# Autodesk Inventor assembly: FE-100 Main Section
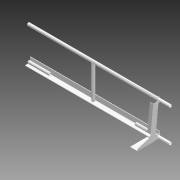
[picture p0: Inventor's stored thumbnail of the model, 180x180]
Saved by Autodesk Inventor 2021 (Build 250183000, 183)
## iProperties
Created: 2021-01-11
Part Number: FE-100 Main Section
Document SubType Name: Assembly
## Documents named in this file (7)
- D:\FIRST\Design\FRC Fields\Generic Field Base\FE-100 Side Wall\FE-110 Main Section\FE-100 Main Section.iam
- D:\FIRST\Design\FRC Fields\Generic Field Base\FE-100 Side Wall\FE-110 Main Section\FE-110-001 Floor L Section.ipt
- D:\FIRST\Design\FRC Fields\Generic Field Base\FE-100 Side Wall\FE-110 Main Section\FE-110-002 Upright Middle Section.ipt
- D:\FIRST\Design\FRC Fields\Generic Field Base\FE-100 Side Wall\FE-110 Main Section\FE-110-003 Top Bar.ipt
- D:\FIRST\Design\FRC Fields\Generic Field Base\FE-100 Side Wall\FE-110 Main Section\FE-110-004 Bottom Side Bar.ipt
- D:\FIRST\Design\FRC Fields\Generic Field Base\FE-100 Side Wall\FE-110 Main Section\FE-110-005 Inside Connector Bar.ipt
- D:\FIRST\Design\FRC Fields\Generic Field Base\FE-100 Side Wall\FE-110 Main Section\FE-110-006 Side Holder.ipt
## Components (8 placed, 6 different names)
1. FE-110-001 Floor L Section:1 — Tangent:1, Mate:2, Flush:1, Angle:1, Tangent:2, Flush:2, Tangent:3, Flush:4
2. FE-110-002 Upright Middle Section:1 — Mate:1, Tangent:1, Mate:2, Mate:3
3. FE-110-003 Top Bar:1 — Mate:3, Flush:1, Angle:1, Mate:4, Flush:3, Mate:5, Mate:6, Mate:7, Insert:1
4. FE-110-004 Bottom Side Bar:1 — Mate:4, Tangent:2, Flush:2, Mate:8, Mate:9, Mate:10, Tangent:4
5. FE-110-004 Bottom Side Bar:2 — Tangent:3, Flush:3, Flush:4
6. FE-110-005 Inside Connector Bar:1 — Mate:5, Mate:6, Mate:7
7. FE-110-005 Inside Connector Bar:2 — Mate:8, Mate:9, Mate:10
8. FE-110-006 Side Holder:1 — Insert:1, Tangent:4
## Relationships (20: Mate 10, Tangent 4, Flush 4, Angle 1, Insert 1)
- Mate:1: FE-110-002 Upright Middle Section:1
- Tangent:1: FE-110-001 Floor L Section:1 ↔ FE-110-002 Upright Middle Section:1
- Mate:2: FE-110-001 Floor L Section:1 ↔ FE-110-002 Upright Middle Section:1
- Mate:3: FE-110-002 Upright Middle Section:1 ↔ FE-110-003 Top Bar:1
- Flush:1: FE-110-001 Floor L Section:1 ↔ FE-110-003 Top Bar:1
- Angle:1 (0 deg): FE-110-001 Floor L Section:1 ↔ FE-110-003 Top Bar:1
- Mate:4: FE-110-003 Top Bar:1 ↔ FE-110-004 Bottom Side Bar:1
- Tangent:2: FE-110-001 Floor L Section:1 ↔ FE-110-004 Bottom Side Bar:1
- Flush:2 (6.35 mm): FE-110-001 Floor L Section:1 ↔ FE-110-004 Bottom Side Bar:1
- Tangent:3: FE-110-001 Floor L Section:1 ↔ FE-110-004 Bottom Side Bar:2
- Flush:3: FE-110-003 Top Bar:1 ↔ FE-110-004 Bottom Side Bar:2
- Flush:4 (6.35 mm): FE-110-001 Floor L Section:1 ↔ FE-110-004 Bottom Side Bar:2
- Mate:5: FE-110-003 Top Bar:1 ↔ FE-110-005 Inside Connector Bar:1
- Mate:6: FE-110-003 Top Bar:1 ↔ FE-110-005 Inside Connector Bar:1
- Mate:7: FE-110-003 Top Bar:1 ↔ FE-110-005 Inside Connector Bar:1
- Mate:8: FE-110-004 Bottom Side Bar:1 ↔ FE-110-005 Inside Connector Bar:2
- Mate:9: FE-110-004 Bottom Side Bar:1 ↔ FE-110-005 Inside Connector Bar:2
- Mate:10: FE-110-004 Bottom Side Bar:1 ↔ FE-110-005 Inside Connector Bar:2
- Insert:1: FE-110-003 Top Bar:1 ↔ FE-110-006 Side Holder:1
- Tangent:4: FE-110-004 Bottom Side Bar:1 ↔ FE-110-006 Side Holder:1
